# Autodesk Inventor assembly: poleStand
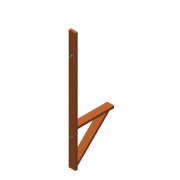
[picture p0: Inventor's stored thumbnail of the model, 180x180]
Saved by Autodesk Inventor 2016 SP2 (Build 200236200, 236)
## iProperties
Created: 2013-12-02
Part Number: poleStand
Document SubType Name: Assembly
Designer: Dave
Author: Dave
## Documents named in this file (7)
- C:\Users\krosie\Google Drive\HERA\hera-cad\support\pole\poleStandVertAssy.iam
- C:\Users\krosie\Google Drive\HERA\hera-cad\support\pole\poleStandVert.ipt
- C:\Users\krosie\Google Drive\HERA\hera-cad\support\pole\poleStandHoriz1.ipt
- C:\Users\krosie\Google Drive\HERA\hera-cad\support\pole\poleStand45.ipt
- C:\Users\krosie\Google Drive\HERA\hera-cad\smallParts\washer_3-8.ipt
- C:\Users\krosie\Google Drive\HERA\hera-cad\smallParts\lagBolt_3-8.ipt
- C:\Users\krosie\Documents\Inventor\Content Center Files\R2016\en-US\AS 2465(1)\AS 2465 - 3_8  UNC(1).ipt
## Components (11 placed, 6 different names)
1. poleStandVert:1 — Insert:1, Insert:4, Insert:5, Flush:7, Flush:8, Mate:4, Mate:6, Mate:8
2. poleStand45:1 — Flush:8, Mate:4, Mate:5
3. poleStandHoriz1:1 — Insert:1, Flush:7, Mate:5
4. washer_3-8:2 — Insert:4, Insert:7
5. washer_3-8:3 — Insert:5, Insert:8
6. lagBolt_3-8:1 — Insert:8, Mate:9
7. lagBolt_3-8:2 — Insert:7, Mate:7, Mate:11, Mate:13
8. washer_3-8:4 — Mate:6, Mate:7, Mate:10
9. washer_3-8:5 — Mate:8, Mate:9
10. AS 2465 - Inch 3/8  UNC:1 — Mate:10, Mate:11, Mate:12
11. AS 2465 - Inch 3/8  UNC:2 — Mate:12, Mate:13
## Relationships (17: Mate 10, Insert 5, Flush 2)
- Insert:1: poleStandVert:1 ↔ poleStandHoriz1:1
- Insert:4: poleStandVert:1 ↔ washer_3-8:2
- Insert:5: poleStandVert:1 ↔ washer_3-8:3
- Insert:7: washer_3-8:2 ↔ lagBolt_3-8:2
- Insert:8: washer_3-8:3 ↔ lagBolt_3-8:1
- Flush:7: poleStandVert:1 ↔ poleStandHoriz1:1
- Flush:8: poleStandVert:1 ↔ poleStand45:1
- Mate:4: poleStandVert:1 ↔ poleStand45:1
- Mate:5: poleStand45:1 ↔ poleStandHoriz1:1
- Mate:6: poleStandVert:1 ↔ washer_3-8:4
- Mate:7: lagBolt_3-8:2 ↔ washer_3-8:4
- Mate:8: poleStandVert:1 ↔ washer_3-8:5
- Mate:9: lagBolt_3-8:1 ↔ washer_3-8:5
- Mate:10: washer_3-8:4 ↔ AS 2465 - Inch 3/8  UNC:1
- Mate:11: lagBolt_3-8:2 ↔ AS 2465 - Inch 3/8  UNC:1
- Mate:12: AS 2465 - Inch 3/8  UNC:1 ↔ AS 2465 - Inch 3/8  UNC:2
- Mate:13: lagBolt_3-8:2 ↔ AS 2465 - Inch 3/8  UNC:2
